# Autodesk Inventor assembly: 200-02-ROCKER-CONNECTOR-ASM-R
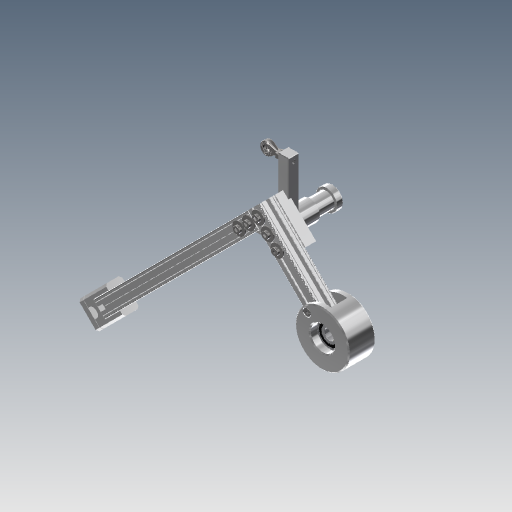
[picture p0: Inventor's stored thumbnail of the model, 512x512]
Saved by Autodesk Inventor 2018.2 (Build 222227000, 227)
## iProperties
Manager: feesmrt
Company: FRANCOR
Created: 2017-12-19
Part Number: 200-02-ROCKER-CONNECTOR-ASM-R
Project: Rescue Robot
Cost Center: -
Material: Generisch
Document SubType Name: Assembly
Designer: feesmrt
Engineer: feesmrt
Authority: feesmrt
Description: Rocker Connector Right Side ASM
Stock Number: 200-02-ROCKER-CONNECTOR-ASM-R
Subject: Rescue Robot
Author: feesmrt
Revision Number: 1
Title: Rocker Connector Right Side ASM
## Documents named in this file (10)
- D:\Programmierung\FRANC0R\CAD\02-Rocker-Bogie-Robot\200-ROCKER-BOGIE\200-02-ROCKER-CONNECTOR-ASM-R.iam
- D:\Programmierung\FRANC0R\CAD\02-Rocker-Bogie-Robot\200-ROCKER-BOGIE\200-20-ROCKER-CONNECTOR\200-20-ROCKER-CONNECTOR-ASM-01.iam
- D:\Programmierung\FRANC0R\CAD\02-Rocker-Bogie-Robot\200-ROCKER-BOGIE\200-30-BOGIE-BEARING\200-30-BOGIE-BEARING-ASM-01.iam
- D:\Programmierung\FRANC0R\CAD\02-Rocker-Bogie-Robot\200-ROCKER-BOGIE\200-50-WHEEL-CONNECTOR\200-50-WHEEL-CONNECTOR-30MM-ASM-01.iam
- D:\Programmierung\FRANC0R\CAD\02-Rocker-Bogie-Robot\200-ROCKER-BOGIE\200-20-ROCKER-CONNECTOR\200-20-ROCKER-CONNECTOR-P-01.ipt
- D:\Programmierung\FRANC0R\CAD\02-Rocker-Bogie-Robot\200-ROCKER-BOGIE\200-20-ROCKER-CONNECTOR\200-20-ROCKER-CONNECTOR-P-02.ipt
- D:\Programmierung\FRANC0R\CAD\02-Rocker-Bogie-Robot\900-COMPONENTS\900-80-WASHERS\900-80-WASHERS-DIN9021-M8.ipt
- D:\Programmierung\FRANC0R\CAD\02-Rocker-Bogie-Robot\900-COMPONENTS\900-40-SCREWS\900-40-SCREWS-DIN7984_M8x45.ipt
- D:\Programmierung\FRANC0R\CAD\02-Rocker-Bogie-Robot\900-COMPONENTS\900-70-ANGLE-JOINTS\900-70-ANGLE-JOINT-DIN648-M8-1.ipt
- D:\Programmierung\FRANC0R\CAD\02-Rocker-Bogie-Robot\900-COMPONENTS\900-41-NUTS\900-41-NUTS-ISO4035-M8.ipt
## Components (18 placed, 9 different names)
1. 200-20-ROCKER-CONNECTOR-ASM-01:1 [sub-assembly] — Passend:4, Fluchtend:3, Fluchtend:6, Passend:8, Fluchtend:7, Passend:35, Winkel:1, Passend:36, Passend:39
2. 200-30-BOGIE-BEARING-ASM-01:1 [sub-assembly] — Passend:10, Passend:13, Passend:14
3. 200-50-WHEEL-CONNECTOR-30MM-ASM-01:1 [sub-assembly] — Passend:6, Passend:7, Fluchtend:5
4. 200-20-ROCKER-CONNECTOR-P-01:1 — Fluchtend:6, Passend:8, Fluchtend:7, Passend:9, Passend:10, Passend:13, Passend:14, Passend:17, Passend:18, Passend:19, Passend:22, Passend:23, Passend:24
5. 200-20-ROCKER-CONNECTOR-P-02:1 — Passend:4, Fluchtend:3, Passend:6, Passend:7, Fluchtend:5, Passend:9, Passend:15, Passend:16, Passend:20, Passend:21
6. 900-80-WASHERS-DIN9021-M8:1 — Passend:15, Passend:20, Passend:25, Passend:34
7. 900-80-WASHERS-DIN9021-M8:2 — Passend:16, Passend:21, Passend:26, Passend:33
8. 900-80-WASHERS-DIN9021-M8:3 — Passend:17, Passend:22, Passend:27, Passend:30
9. 900-80-WASHERS-DIN9021-M8:4 — Passend:18, Passend:23, Passend:28, Passend:31
10. 900-80-WASHERS-DIN9021-M8:5 — Passend:19, Passend:24, Passend:29, Passend:32
11. 900-40-SCREWS-DIN7984_M8x45:1 — Passend:25, Passend:34
12. 900-40-SCREWS-DIN7984_M8x45:2 — Passend:26, Passend:33
13. 900-40-SCREWS-DIN7984_M8x45:3 — Passend:27, Passend:30
14. 900-40-SCREWS-DIN7984_M8x45:4 — Passend:28, Passend:31
15. 900-40-SCREWS-DIN7984_M8x45:5 — Passend:29, Passend:32
16. 900-70-ANGLE-JOINT-DIN648-M8-1:1 — Passend:35, Winkel:1, Passend:36, Passend:37, Passend:38
17. 900-41-NUTS-ISO4035-M8:1 — Passend:38, Passend:40
18. 900-41-NUTS-ISO4035-M8:2 — Passend:37, Passend:39, Passend:40
## Relationships (39: Mate 34, Flush 4, Angle 1)
- Passend:4 [Mate]: 200-20-ROCKER-CONNECTOR-ASM-01:1 ↔ 200-20-ROCKER-CONNECTOR-P-02:1
- Fluchtend:3 [Flush]: 200-20-ROCKER-CONNECTOR-ASM-01:1 ↔ 200-20-ROCKER-CONNECTOR-P-02:1
- Passend:6 [Mate]: 200-50-WHEEL-CONNECTOR-30MM-ASM-01:1 ↔ 200-20-ROCKER-CONNECTOR-P-02:1
- Passend:7 [Mate]: 200-50-WHEEL-CONNECTOR-30MM-ASM-01:1 ↔ 200-20-ROCKER-CONNECTOR-P-02:1
- Fluchtend:5 [Flush]: 200-50-WHEEL-CONNECTOR-30MM-ASM-01:1 ↔ 200-20-ROCKER-CONNECTOR-P-02:1
- Fluchtend:6 [Flush]: 200-20-ROCKER-CONNECTOR-ASM-01:1 ↔ 200-20-ROCKER-CONNECTOR-P-01:1
- Passend:8 [Mate]: 200-20-ROCKER-CONNECTOR-ASM-01:1 ↔ 200-20-ROCKER-CONNECTOR-P-01:1
- Fluchtend:7 [Flush]: 200-20-ROCKER-CONNECTOR-ASM-01:1 ↔ 200-20-ROCKER-CONNECTOR-P-01:1
- Passend:9 [Mate]: 200-20-ROCKER-CONNECTOR-P-01:1 ↔ 200-20-ROCKER-CONNECTOR-P-02:1
- Passend:10 [Mate]: 200-30-BOGIE-BEARING-ASM-01:1 ↔ 200-20-ROCKER-CONNECTOR-P-01:1
- Passend:13 [Mate]: 200-30-BOGIE-BEARING-ASM-01:1 ↔ 200-20-ROCKER-CONNECTOR-P-01:1
- Passend:14 [Mate]: 200-30-BOGIE-BEARING-ASM-01:1 ↔ 200-20-ROCKER-CONNECTOR-P-01:1
- Passend:15 [Mate]: 200-20-ROCKER-CONNECTOR-P-02:1 ↔ 900-80-WASHERS-DIN9021-M8:1
- Passend:16 [Mate]: 200-20-ROCKER-CONNECTOR-P-02:1 ↔ 900-80-WASHERS-DIN9021-M8:2
- Passend:17 [Mate]: 200-20-ROCKER-CONNECTOR-P-01:1 ↔ 900-80-WASHERS-DIN9021-M8:3
- Passend:18 [Mate]: 200-20-ROCKER-CONNECTOR-P-01:1 ↔ 900-80-WASHERS-DIN9021-M8:4
- Passend:19 [Mate]: 200-20-ROCKER-CONNECTOR-P-01:1 ↔ 900-80-WASHERS-DIN9021-M8:5
- Passend:20 [Mate]: 200-20-ROCKER-CONNECTOR-P-02:1 ↔ 900-80-WASHERS-DIN9021-M8:1
- Passend:21 [Mate]: 200-20-ROCKER-CONNECTOR-P-02:1 ↔ 900-80-WASHERS-DIN9021-M8:2
- Passend:22 [Mate]: 200-20-ROCKER-CONNECTOR-P-01:1 ↔ 900-80-WASHERS-DIN9021-M8:3
- Passend:23 [Mate]: 200-20-ROCKER-CONNECTOR-P-01:1 ↔ 900-80-WASHERS-DIN9021-M8:4
- Passend:24 [Mate]: 200-20-ROCKER-CONNECTOR-P-01:1 ↔ 900-80-WASHERS-DIN9021-M8:5
- Passend:25 [Mate]: 900-80-WASHERS-DIN9021-M8:1 ↔ 900-40-SCREWS-DIN7984_M8x45:1
- Passend:26 [Mate]: 900-80-WASHERS-DIN9021-M8:2 ↔ 900-40-SCREWS-DIN7984_M8x45:2
- Passend:27 [Mate]: 900-80-WASHERS-DIN9021-M8:3 ↔ 900-40-SCREWS-DIN7984_M8x45:3
- Passend:28 [Mate]: 900-80-WASHERS-DIN9021-M8:4 ↔ 900-40-SCREWS-DIN7984_M8x45:4
- Passend:29 [Mate]: 900-80-WASHERS-DIN9021-M8:5 ↔ 900-40-SCREWS-DIN7984_M8x45:5
- Passend:30 [Mate]: 900-80-WASHERS-DIN9021-M8:3 ↔ 900-40-SCREWS-DIN7984_M8x45:3
- Passend:31 [Mate]: 900-80-WASHERS-DIN9021-M8:4 ↔ 900-40-SCREWS-DIN7984_M8x45:4
- Passend:32 [Mate]: 900-80-WASHERS-DIN9021-M8:5 ↔ 900-40-SCREWS-DIN7984_M8x45:5
- Passend:33 [Mate]: 900-80-WASHERS-DIN9021-M8:2 ↔ 900-40-SCREWS-DIN7984_M8x45:2
- Passend:34 [Mate]: 900-80-WASHERS-DIN9021-M8:1 ↔ 900-40-SCREWS-DIN7984_M8x45:1
- Passend:35 [Mate]: 200-20-ROCKER-CONNECTOR-ASM-01:1 ↔ 900-70-ANGLE-JOINT-DIN648-M8-1:1
- Winkel:1 [Angle] (0 deg): 200-20-ROCKER-CONNECTOR-ASM-01:1 ↔ 900-70-ANGLE-JOINT-DIN648-M8-1:1
- Passend:36 [Mate] (10 mm): 200-20-ROCKER-CONNECTOR-ASM-01:1 ↔ 900-70-ANGLE-JOINT-DIN648-M8-1:1
- Passend:37 [Mate]: 900-70-ANGLE-JOINT-DIN648-M8-1:1 ↔ 900-41-NUTS-ISO4035-M8:2
- Passend:38 [Mate]: 900-70-ANGLE-JOINT-DIN648-M8-1:1 ↔ 900-41-NUTS-ISO4035-M8:1
- Passend:39 [Mate]: 200-20-ROCKER-CONNECTOR-ASM-01:1 ↔ 900-41-NUTS-ISO4035-M8:2
- Passend:40 [Mate]: 900-41-NUTS-ISO4035-M8:1 ↔ 900-41-NUTS-ISO4035-M8:2
